# Autodesk Inventor assembly: 前後直動
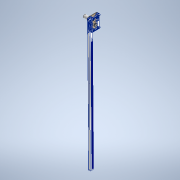
[picture p0: Inventor's stored thumbnail of the model, 180x180]
Saved by Autodesk Inventor 2020.3 (Build 243373000, 373)
## iProperties
Created: 2020-07-05
Part Number: 前後直動
Document SubType Name: Assembly
Designer: totot
Mass: 1557.98 g
Surface Area: 5821.56 cm^2
Volume: 677.992 cm^3
Density: 2.29793 g/cm^3
Author: totot
## Documents named in this file (10)
- D:\mysvn\ロボコン\キャチロボ\キャチロボ設計図\ロボット\前後直動\前後直動.iam
- D:\mysvn\ロボコン\キャチロボ\キャチロボ設計図\ロボット\ハンド\12ｘ12_1.ipt
- D:\mysvn\ロボコン\キャチロボ\キャチロボ設計図\ロボット\共有パーツ\DR1-2000_On2.ipt
- D:\mysvn\ロボコン\キャチロボ\キャチロボ設計図\ロボット\前後直動\前後直動12x12_2.ipt
- D:\mysvn\ロボコン\キャチロボ\キャチロボ設計図\ロボット\前後直動\前後直動12x12_3.ipt
- D:\mysvn\ロボコン\キャチロボ\キャチロボ設計図\ロボット\前後直動\前後直動12x12_4.ipt
- D:\mysvn\ロボコン\キャチロボ\キャチロボ設計図\ロボット\共有パーツ\RS_380.ipt
- D:\mysvn\ロボコン\キャチロボ\キャチロボ設計図\ロボット\前後直動\前後直動9x9x24.ipt
- D:\mysvn\ロボコン\キャチロボ\キャチロボ設計図\ロボット\共有パーツ\ポテンションメーター_BI-7284.ipt
- D:\mysvn\ロボコン\キャチロボ\キャチロボ設計図\ロボット\共有パーツ\PS1-20_On.ipt
## Components (14 placed, 9 different names)
1. 12ｘ12_1:1 — 挿入:1, 挿入:2, 挿入:3, 挿入:5, 挿入:10, 挿入:14, 挿入:16, 挿入:18, メイト:1, フラッシュ:1, フラッシュ:2
2. DR1-2000_On2:1 — メイト:1, フラッシュ:1, フラッシュ:2
3. 前後直動t5_1 — 挿入:15, 挿入:16, 挿入:17, 挿入:18, 挿入:19, 挿入:20, 挿入:22, 挿入:23
4. RS_380:1 — 挿入:22, 挿入:23
5. 12ｘ12_1:2 — 挿入:1, 挿入:2
6. 前後直動12x12_3:1 — 挿入:7, 挿入:8, 挿入:9, 挿入:12, 挿入:15, 挿入:17, 挿入:19
7. 前後直動12x12_2:1 — 挿入:3, 挿入:4, 挿入:6, 挿入:7
8. 前後直動12x12_2:2 — 挿入:11, 挿入:12, 挿入:13, 挿入:14
9. 前後直動9x9x24:1 — 挿入:9, 挿入:11
10. 前後直動9x9x24:2 — 挿入:6, 挿入:8
11. 前後直動9x9x24:3 — 挿入:10, 挿入:13
12. 前後直動9x9x24:4 — 挿入:4, 挿入:5
13. ポテンションメーター_BI-7284:1 — 挿入:20, 挿入:21
14. PS1-20_On:1 — 挿入:21
## Relationships (26: Insert 23, Flush 2, Mate 1)
- 挿入:1 [Insert]: 12ｘ12_1:1 ↔ 12ｘ12_1:2
- 挿入:2 [Insert]: 12ｘ12_1:1 ↔ 12ｘ12_1:2
- 挿入:3 [Insert]: 12ｘ12_1:1 ↔ 前後直動12x12_2:1
- 挿入:4 [Insert]: 前後直動12x12_2:1 ↔ 前後直動9x9x24:4
- 挿入:5 [Insert]: 12ｘ12_1:1 ↔ 前後直動9x9x24:4
- 挿入:6 [Insert]: 前後直動12x12_2:1 ↔ 前後直動9x9x24:2
- 挿入:7 [Insert]: 前後直動12x12_3:1 ↔ 前後直動12x12_2:1
- 挿入:8 [Insert]: 前後直動12x12_3:1 ↔ 前後直動9x9x24:2
- 挿入:9 [Insert]: 前後直動12x12_3:1 ↔ 前後直動9x9x24:1
- 挿入:10 [Insert]: 12ｘ12_1:1 ↔ 前後直動9x9x24:3
- 挿入:11 [Insert]: 前後直動12x12_2:2 ↔ 前後直動9x9x24:1
- 挿入:12 [Insert]: 前後直動12x12_3:1 ↔ 前後直動12x12_2:2
- 挿入:13 [Insert]: 前後直動12x12_2:2 ↔ 前後直動9x9x24:3
- 挿入:14 [Insert]: 12ｘ12_1:1 ↔ 前後直動12x12_2:2
- 挿入:15 [Insert]: 前後直動t5_1 ↔ 前後直動12x12_3:1
- 挿入:16 [Insert]: 12ｘ12_1:1 ↔ 前後直動t5_1
- 挿入:17 [Insert]: 前後直動t5_1 ↔ 前後直動12x12_3:1
- 挿入:18 [Insert]: 12ｘ12_1:1 ↔ 前後直動t5_1
- 挿入:19 [Insert]: 前後直動t5_1 ↔ 前後直動12x12_3:1
- 挿入:20 [Insert]: 前後直動t5_1 ↔ ポテンションメーター_BI-7284:1
- 挿入:21 [Insert] (-10 mm): ポテンションメーター_BI-7284:1 ↔ PS1-20_On:1
- 挿入:22 [Insert]: 前後直動t5_1 ↔ RS_380:1
- 挿入:23 [Insert]: 前後直動t5_1 ↔ RS_380:1
- メイト:1 [Mate]: 12ｘ12_1:1 ↔ DR1-2000_On2:1
- フラッシュ:1 [Flush] (-2 mm): 12ｘ12_1:1 ↔ DR1-2000_On2:1
- フラッシュ:2 [Flush] (-10 mm): 12ｘ12_1:1 ↔ DR1-2000_On2:1
